# Autodesk Inventor assembly: サス
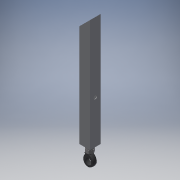
[picture p0: Inventor's stored thumbnail of the model, 180x180]
Saved by Autodesk Inventor 2018 (Build 220112000, 112)
## iProperties
Created: 2017-09-07
Part Number: サス
Material: 一般
Document SubType Name: Assembly
Designer: Kosei
Author: Kosei
## Documents named in this file (5)
- C:\Users\mura5\Documents\RBBR\cart\Rod1.iam
- C:\Users\mura5\Documents\RBBR\cart\Pipe1.ipt
- C:\Users\mura5\Documents\RBBR\cart\ナット蓋.ipt
- C:\Users\mura5\Documents\RBBR\cart\hn1_12.ipt
- C:\Users\mura5\Documents\RBBR\cart\iko_POS_12\AIS2014\POS 12 Body.ipt
## Components (5 placed, 4 different names)
1. Pipe1:1 — リジッド:4
2. ナット蓋:1 — リジッド:4, リジッド:5, 回転:1
3. hn1_12:1 — リジッド:5, 円柱状:1, リジッド:6
4. hn1_12:2 — リジッド:6
5. POS 12 Body:1 — 円柱状:1, 回転:1
## Relationships (5: WeldJoint 3, CylindricalJoint 1, RevoluteJoint 1)
- リジッド:4 [WeldJoint]: Pipe1:1 ↔ ナット蓋:1
- リジッド:5 [WeldJoint]: ナット蓋:1 ↔ hn1_12:1
- 円柱状:1 [CylindricalJoint]: hn1_12:1 ↔ POS 12 Body:1
- リジッド:6 [WeldJoint]: hn1_12:1 ↔ hn1_12:2
- 回転:1 [RevoluteJoint] (12 mm): ナット蓋:1 ↔ POS 12 Body:1
